# Autodesk Inventor assembly: Aerosky MC4230 630KV
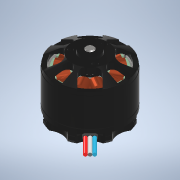
[picture p0: Inventor's stored thumbnail of the model, 180x180]
Saved by Autodesk Inventor 2022 (Build 260153000, 153)
## iProperties
Created: 2022-07-25
Part Number: Aerosky MC4230 630KV
Document SubType Name: Assembly
Designer: Nathan Cai
Author: Nathan Cai
## Documents named in this file (3)
- C:\Users\Nathan Cai\Documents\Inventor\Asorted Parts\Aerosky MC4230 630KV\Aerosky MC4230 630KV.iam
- C:\Users\Nathan Cai\Documents\Inventor\Asorted Parts\Aerosky MC4230 630KV\CAN.iam
- C:\Users\Nathan Cai\Documents\Inventor\Asorted Parts\Aerosky MC4230 630KV\BASE.iam
## Components (2 placed, 2 different names)
1. CAN:1 [sub-assembly] — Mate:1, Mate:2
2. BASE:1 [sub-assembly] — Mate:1, Mate:2
## Relationships (2: Mate 2)
- Mate:1: CAN:1 ↔ BASE:1
- Mate:2: CAN:1 ↔ BASE:1
